# Autodesk Inventor assembly: extension arm
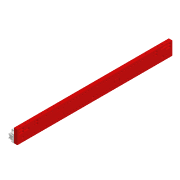
[picture p0: Inventor's stored thumbnail of the model, 180x180]
Saved by Autodesk Inventor 2020 (Build 240168000, 168)
## iProperties
Created: 2019-12-12
Part Number: extension arm
Document SubType Name: Assembly
Designer: ball
Author: ball
## Documents named in this file (4)
- C:\FTC\FTC8863CAD\2019 Robot\Delivery\extension arm\extension arm top.iam
- C:\FTC\FTC8863CAD\2019 Robot\Delivery\extension arm\Coupler extension arm short.ipt
- C:\FTC\FTC8863CAD\Misumi\SAR340\SAR340 offset 10 mm.iam
- C:\FTC\FTC8863CAD\2019 Robot\Delivery\extension arm\Coupler extension arm motor.ipt
## Components (3 placed, 3 different names)
1. SAR340 offset 10 mm:1 [sub-assembly] — Mate:1, Mate:2, Mate:3, Mate:4, Mate:5, Flush:1
2. Coupler extension arm motor:1 — Mate:1, Mate:2, Mate:3
3. Coupler extension arm short:1 — Mate:4, Mate:5, Flush:1
## Relationships (6: Mate 5, Flush 1)
- Mate:1: SAR340 offset 10 mm:1 ↔ Coupler extension arm motor:1
- Mate:2: SAR340 offset 10 mm:1 ↔ Coupler extension arm motor:1
- Mate:3: SAR340 offset 10 mm:1 ↔ Coupler extension arm motor:1
- Mate:4: SAR340 offset 10 mm:1 ↔ Coupler extension arm short:1
- Mate:5: SAR340 offset 10 mm:1 ↔ Coupler extension arm short:1
- Flush:1: SAR340 offset 10 mm:1 ↔ Coupler extension arm short:1
